# Autodesk Inventor assembly: 조립품1
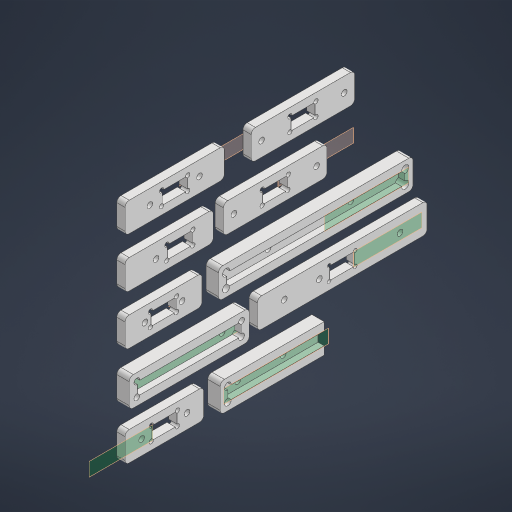
[picture p0: Inventor's stored thumbnail of the model, 512x512]
Saved by Autodesk Inventor 2024.3 (Build 283343000, 343)
## iProperties
Created: 2024-09-11
Part Number: 조립품1
Document SubType Name: Assembly
Designer: ASUS
Author: ASUS
## Documents named in this file (11)
- C:\Users\ASUS\Desktop\19th_Freshmen\ZIG\Zig_Assemble.iam
- C:\Users\ASUS\Desktop\19th_Freshmen\ZIG\zig1.ipt
- C:\Users\ASUS\Desktop\19th_Freshmen\ZIG\zig2.ipt
- C:\Users\ASUS\Desktop\19th_Freshmen\ZIG\zig3.ipt
- C:\Users\ASUS\Desktop\19th_Freshmen\ZIG\zig4.ipt
- C:\Users\ASUS\Desktop\19th_Freshmen\ZIG\zig5.ipt
- C:\Users\ASUS\Desktop\19th_Freshmen\ZIG\zig6.ipt
- C:\Users\ASUS\Desktop\19th_Freshmen\ZIG\zig7.ipt
- C:\Users\ASUS\Desktop\19th_Freshmen\ZIG\zig8.ipt
- C:\Users\ASUS\Desktop\19th_Freshmen\ZIG\zig9.ipt
- C:\Users\ASUS\Desktop\19th_Freshmen\ZIG\zig10.ipt
## Components (10 placed, 10 different names)
1. zig1:1 — 플러쉬:1, 플러쉬:2, 메이트:1, 플러쉬:3, 플러쉬:4, 메이트:11, 플러쉬:22
2. zig2:1 — 메이트:1, 플러쉬:3, 플러쉬:4, 플러쉬:5, 플러쉬:6, 메이트:2, 메이트:13, 플러쉬:24
3. zig3:1 — 플러쉬:1, 플러쉬:2, 플러쉬:5, 플러쉬:6, 메이트:2, 플러쉬:7, 메이트:3, 플러쉬:8, 플러쉬:9, 플러쉬:10, 메이트:12, 플러쉬:23
4. zig4:1 — 플러쉬:7, 메이트:3, 플러쉬:8, 메이트:4, 플러쉬:25, 메이트:14
5. zig5:1 — 플러쉬:9, 플러쉬:10, 메이트:4, 플러쉬:11, 메이트:15
6. zig6:1 — 플러쉬:11, 플러쉬:13, 플러쉬:17, 메이트:11, 플러쉬:22
7. zig8:1 — 플러쉬:13, 플러쉬:16, 메이트:13, 플러쉬:24
8. zig9:1 — 플러쉬:16, 플러쉬:19, 메이트:10, 플러쉬:25, 메이트:14
9. zig7:1 — 플러쉬:17, 메이트:12, 플러쉬:23
10. zig10:1 — 플러쉬:19, 메이트:10, 메이트:15
## Relationships (29: Flush 19, Mate 10)
- 플러쉬:1 [Flush]: zig1:1 ↔ zig3:1
- 플러쉬:2 [Flush]: zig1:1 ↔ zig3:1
- 메이트:1 [Mate] (10 mm): zig1:1 ↔ zig2:1
- 플러쉬:3 [Flush]: zig1:1 ↔ zig2:1
- 플러쉬:4 [Flush]: zig1:1 ↔ zig2:1
- 플러쉬:5 [Flush]: zig2:1 ↔ zig3:1
- 플러쉬:6 [Flush]: zig2:1 ↔ zig3:1
- 메이트:2 [Mate] (10 mm): zig2:1 ↔ zig3:1
- 플러쉬:7 [Flush]: zig3:1 ↔ zig4:1
- 메이트:3 [Mate] (10 mm): zig3:1 ↔ zig4:1
- 플러쉬:8 [Flush]: zig3:1 ↔ zig4:1
- 플러쉬:9 [Flush]: zig3:1 ↔ zig5:1
- 플러쉬:10 [Flush]: zig3:1 ↔ zig5:1
- 메이트:4 [Mate] (10 mm): zig4:1 ↔ zig5:1
- 플러쉬:11 [Flush]: zig5:1 ↔ zig6:1
- 플러쉬:13 [Flush]: zig6:1 ↔ zig8:1
- 플러쉬:16 [Flush]: zig8:1 ↔ zig9:1
- 플러쉬:17 [Flush]: zig6:1 ↔ zig7:1
- 플러쉬:19 [Flush]: zig9:1 ↔ zig10:1
- 메이트:10 [Mate] (10 mm): zig9:1 ↔ zig10:1
- 메이트:11 [Mate] (13 mm): zig1:1 ↔ zig6:1
- 플러쉬:22 [Flush]: zig1:1 ↔ zig6:1
- 메이트:12 [Mate] (6 mm): zig3:1 ↔ zig7:1
- 플러쉬:23 [Flush]: zig3:1 ↔ zig7:1
- 메이트:13 [Mate] (5 mm): zig2:1 ↔ zig8:1
- 플러쉬:24 [Flush]: zig2:1 ↔ zig8:1
- 플러쉬:25 [Flush]: zig4:1 ↔ zig9:1
- 메이트:14 [Mate] (6 mm): zig4:1 ↔ zig9:1
- 메이트:15 [Mate] (6 mm): zig5:1 ↔ zig10:1
